# Autodesk Inventor assembly: Drone V2
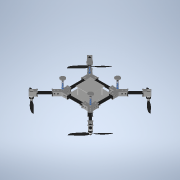
[picture p0: Inventor's stored thumbnail of the model, 180x180]
Saved by Autodesk Inventor 2022 (Build 260153000, 153)
## iProperties
Created: 2022-02-02
Part Number: Drone V2
Document SubType Name: Assembly
Designer: ultra
Author: ultra
## Documents named in this file (7)
- C:\Users\ultra\Desktop\Github\RASA-Drone\CAD Files\Drone\Drone V2.iam
- C:\Users\ultra\Desktop\Github\RASA-Drone\CAD Files\Drone\Tube.ipt
- C:\Users\ultra\Desktop\Github\RASA-Drone\CAD Files\Drone\Subframe V1.iam
- C:\Users\ultra\Desktop\Github\RASA-Drone\CAD Files\Drone\Frame.ipt
- C:\Users\ultra\Desktop\Github\RASA-Drone\CAD Files\Drone\2inStandoff.ipt
- C:\Users\ultra\Desktop\Github\RASA-Drone\CAD Files\Drone\1.5Standoff.ipt
- C:\Users\ultra\Desktop\Github\RASA-Drone\CAD Files\Drone\Plate.ipt
## Components (19 placed, 6 different names)
1. Tube:2 — Insert:5, Insert:9
2. Tube:10 — Insert:1, Insert:8
3. Subframe V1:1 [sub-assembly] — Insert:8, Insert:9
4. Tube:12 — Insert:3, Insert:4
5. Subframe V1:2 [sub-assembly] — Flush:1, Flush:2, Insert:1, Insert:3, Mate:1
6. Tube:13 — Insert:6, Insert:7
7. Subframe V1:3 [sub-assembly] — Insert:5, Insert:6
8. Subframe V1:4 [sub-assembly] — Flush:1, Flush:2, Insert:4, Insert:7
9. Frame:1 — Mate:1, Insert:10, Insert:11, Insert:12, Insert:13, Insert:14, Insert:15, Insert:16, Insert:17
10. 2inStandoff:1 — Insert:10, Insert:20
11. 2inStandoff:2 — Insert:11
12. 2inStandoff:3 — Insert:12
13. 2inStandoff:4 — Insert:13, Insert:21
14. 1.5Standoff:1 — Insert:17, Insert:18
15. 1.5Standoff:2 — Insert:16, Insert:19
16. 1.5Standoff:3 — Insert:15
17. 1.5Standoff:4 — Insert:14
18. Plate:1 — Insert:18, Insert:19
19. Plate:2 — Insert:20, Insert:21
## Relationships (23: Insert 20, Flush 2, Mate 1)
- Flush:1: Subframe V1:2 ↔ Subframe V1:4
- Flush:2: Subframe V1:2 ↔ Subframe V1:4
- Insert:1: Tube:10 ↔ Subframe V1:2
- Insert:3: Tube:12 ↔ Subframe V1:2
- Insert:4: Tube:12 ↔ Subframe V1:4
- Insert:5: Tube:2 ↔ Subframe V1:3
- Insert:6: Tube:13 ↔ Subframe V1:3
- Insert:7: Tube:13 ↔ Subframe V1:4
- Insert:8: Tube:10 ↔ Subframe V1:1
- Insert:9: Tube:2 ↔ Subframe V1:1
- Mate:1: Subframe V1:2 ↔ Frame:1
- Insert:10: Frame:1 ↔ 2inStandoff:1
- Insert:11: Frame:1 ↔ 2inStandoff:2
- Insert:12: Frame:1 ↔ 2inStandoff:3
- Insert:13: Frame:1 ↔ 2inStandoff:4
- Insert:14: Frame:1 ↔ 1.5Standoff:4
- Insert:15: Frame:1 ↔ 1.5Standoff:3
- Insert:16: Frame:1 ↔ 1.5Standoff:2
- Insert:17: Frame:1 ↔ 1.5Standoff:1
- Insert:18: 1.5Standoff:1 ↔ Plate:1
- Insert:19: 1.5Standoff:2 ↔ Plate:1
- Insert:20: 2inStandoff:1 ↔ Plate:2
- Insert:21: 2inStandoff:4 ↔ Plate:2
